# Autodesk Inventor assembly: Tower Pro MG90S Micro servo
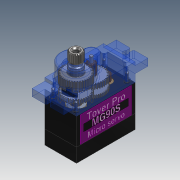
[picture p0: Inventor's stored thumbnail of the model, 180x180]
Saved by Autodesk Inventor 2017 (Build 210142000, 142)
## iProperties
Created: 2018-08-23
Part Number: Tower Pro MG90S Micro servo
Document SubType Name: Assembly
Designer: Shepelev
Mass: 15.118 g
Surface Area: 91.105 cm^2
Volume: 4.7278 cm^3
Density: 3.19769 g/cm^3
Author: Shepelev
## Documents named in this file (14)
- C:\Users\Anton\Desktop\Tower Pro MG90S Micro servo\Tower Pro MG90S Micro servo.iam
- C:\Users\Anton\Desktop\Tower Pro MG90S Micro servo\основание крпуса редуктора.ipt
- C:\Users\Anton\Desktop\Tower Pro MG90S Micro servo\Вал промежуточный.ipt
- C:\Users\Anton\Desktop\Tower Pro MG90S Micro servo\Вал последний с чем то.ipt
- C:\Users\Anton\Desktop\Tower Pro MG90S Micro servo\Моторчик.ipt
- C:\Users\Anton\Desktop\Tower Pro MG90S Micro servo\Tower Pro MG90S Micro servo\Мастер проектирования\Цилиндрическое зубчатое зацепление2.iam
- C:\Users\Anton\Desktop\Tower Pro MG90S Micro servo\Tower Pro MG90S Micro servo\Мастер проектирования\Цилиндрическое зубчатое зацепление3.iam
- C:\Users\Anton\Desktop\Tower Pro MG90S Micro servo\Tower Pro MG90S Micro servo\Мастер проектирования\Цилиндрическое зубчатое зацепление4.iam
- C:\Users\Anton\Desktop\Tower Pro MG90S Micro servo\Tower Pro MG90S Micro servo\Мастер проектирования\Цилиндрическое зубчатое зацепление5.iam
- C:\Users\Anton\Desktop\Tower Pro MG90S Micro servo\ограничитель.ipt
- C:\Users\Anton\Desktop\Tower Pro MG90S Micro servo\Крышка корпуса.ipt
- C:\Users\Anton\Desktop\Tower Pro MG90S Micro servo\Крышка корпуса задняя.ipt
- C:\Users\Anton\Desktop\Tower Pro MG90S Micro servo\Длинный винт.ipt
- C:\Users\Anton\Desktop\Tower Pro MG90S Micro servo\Этикетка.ipt
## Components (17 placed, 10 different names)
1. основание крпуса редуктора:1 — Совмещение:1, Заподлицо:1, Заподлицо:2, Вставка:1, Вставка:2, Вставка:3, Совмещение:2, Совмещение:4, Совмещение:6, Совмещение:23, Совмещение:24, Совмещение:25, Совмещение:26, Совмещение:27, Совмещение:28, Совмещение:29, Заподлицо:5, Заподлицо:6, Заподлицо:7, Заподлицо:8, Совмещение:30
2. Вал промежуточный:1 — Вставка:1, Заподлицо:3, Совмещение:5, Совмещение:7, Совмещение:14, Совмещение:18
3. Вал последний с чем то:1 — Вставка:2, Заподлицо:4, Совмещение:9, Совмещение:12, С поворотом:1
4. Моторчик:1 — Вставка:3, Совмещение:2, Совмещение:3
5. Цилиндрическое зубчатое зацепление:2 [sub-assembly] — Совмещение:3, Совмещение:4, Совмещение:5, Совмещение:6, Совмещение:8, Совмещение:10, Совмещение:11
6. Цилиндрическое зубчатое зацепление:3 [sub-assembly] — Совмещение:7, Совмещение:8, Совмещение:9, Совмещение:10, Совмещение:11, Совмещение:13, Совмещение:15, Совмещение:16
7. Цилиндрическое зубчатое зацепление:4 [sub-assembly] — Совмещение:12, Совмещение:13, Совмещение:14, Совмещение:15, Совмещение:16, Вставка:8, Совмещение:17, Совмещение:19
8. Цилиндрическое зубчатое зацепление:5 [sub-assembly] — Совмещение:18, Совмещение:19, Совмещение:20, Совмещение:21, Совмещение:22
9. ограничитель:2 — Вставка:8, Совмещение:17, С поворотом:1, Совмещение:20, Совмещение:21, Совмещение:22
10. Крышка корпуса:1 — Совмещение:23, Совмещение:24, Совмещение:25
11. Крышка корпуса задняя:1 — Совмещение:26, Совмещение:27, Совмещение:28, Вставка:9, Вставка:10, Вставка:11, Вставка:12
12. Длинный винт:1 — Вставка:9
13. Длинный винт:2 — Вставка:11
14. Длинный винт:3 — Вставка:10
15. Длинный винт:4 — Вставка:12
16. Этикетка:1 — Совмещение:29, Заподлицо:5, Заподлицо:6
17. Этикетка:2 — Заподлицо:7, Заподлицо:8, Совмещение:30
## Relationships (47: Mate 30, Flush 8, Insert 8, RevoluteJoint 1)
- Совмещение:1 [Mate]: основание крпуса редуктора:1
- Заподлицо:1 [Flush]: основание крпуса редуктора:1
- Заподлицо:2 [Flush]: основание крпуса редуктора:1
- Вставка:1 [Insert]: основание крпуса редуктора:1 ↔ Вал промежуточный:1
- Заподлицо:3 [Flush]: Вал промежуточный:1
- Вставка:2 [Insert]: основание крпуса редуктора:1 ↔ Вал последний с чем то:1
- Заподлицо:4 [Flush]: Вал последний с чем то:1
- Вставка:3 [Insert]: основание крпуса редуктора:1 ↔ Моторчик:1
- Совмещение:2 [Mate]: основание крпуса редуктора:1 ↔ Моторчик:1
- Совмещение:3 [Mate]: Моторчик:1 ↔ Цилиндрическое зубчатое зацепление:2
- Совмещение:4 [Mate]: основание крпуса редуктора:1 ↔ Цилиндрическое зубчатое зацепление:2
- Совмещение:5 [Mate]: Вал промежуточный:1 ↔ Цилиндрическое зубчатое зацепление:2
- Совмещение:6 [Mate]: основание крпуса редуктора:1 ↔ Цилиндрическое зубчатое зацепление:2
- Совмещение:7 [Mate]: Вал промежуточный:1 ↔ Цилиндрическое зубчатое зацепление:3
- Совмещение:8 [Mate]: Цилиндрическое зубчатое зацепление:2 ↔ Цилиндрическое зубчатое зацепление:3
- Совмещение:9 [Mate]: Вал последний с чем то:1 ↔ Цилиндрическое зубчатое зацепление:3
- Совмещение:10 [Mate]: Цилиндрическое зубчатое зацепление:2 ↔ Цилиндрическое зубчатое зацепление:3
- Совмещение:11 [Mate]: Цилиндрическое зубчатое зацепление:2 ↔ Цилиндрическое зубчатое зацепление:3
- Совмещение:12 [Mate]: Вал последний с чем то:1 ↔ Цилиндрическое зубчатое зацепление:4
- Совмещение:13 [Mate]: Цилиндрическое зубчатое зацепление:3 ↔ Цилиндрическое зубчатое зацепление:4
- Совмещение:14 [Mate]: Вал промежуточный:1 ↔ Цилиндрическое зубчатое зацепление:4
- Совмещение:15 [Mate]: Цилиндрическое зубчатое зацепление:3 ↔ Цилиндрическое зубчатое зацепление:4
- Совмещение:16 [Mate]: Цилиндрическое зубчатое зацепление:3 ↔ Цилиндрическое зубчатое зацепление:4
- Вставка:8 [Insert]: Цилиндрическое зубчатое зацепление:4 ↔ ограничитель:2
- Совмещение:17 [Mate]: Цилиндрическое зубчатое зацепление:4 ↔ ограничитель:2
- С поворотом:1 [RevoluteJoint] (0.4 mm): Вал последний с чем то:1 ↔ ограничитель:2
- Совмещение:18 [Mate]: Вал промежуточный:1 ↔ Цилиндрическое зубчатое зацепление:5
- Совмещение:19 [Mate]: Цилиндрическое зубчатое зацепление:4 ↔ Цилиндрическое зубчатое зацепление:5
- Совмещение:20 [Mate]: Цилиндрическое зубчатое зацепление:5 ↔ ограничитель:2
- Совмещение:21 [Mate]: Цилиндрическое зубчатое зацепление:5 ↔ ограничитель:2
- Совмещение:22 [Mate]: Цилиндрическое зубчатое зацепление:5 ↔ ограничитель:2
- Совмещение:23 [Mate]: основание крпуса редуктора:1 ↔ Крышка корпуса:1
- Совмещение:24 [Mate]: основание крпуса редуктора:1 ↔ Крышка корпуса:1
- Совмещение:25 [Mate]: основание крпуса редуктора:1 ↔ Крышка корпуса:1
- Совмещение:26 [Mate]: основание крпуса редуктора:1 ↔ Крышка корпуса задняя:1
- Совмещение:27 [Mate]: основание крпуса редуктора:1 ↔ Крышка корпуса задняя:1
- Совмещение:28 [Mate]: основание крпуса редуктора:1 ↔ Крышка корпуса задняя:1
- Вставка:9 [Insert]: Крышка корпуса задняя:1 ↔ Длинный винт:1
- Вставка:10 [Insert]: Крышка корпуса задняя:1 ↔ Длинный винт:3
- Вставка:11 [Insert]: Крышка корпуса задняя:1 ↔ Длинный винт:2
- Вставка:12 [Insert]: Крышка корпуса задняя:1 ↔ Длинный винт:4
- Совмещение:29 [Mate]: основание крпуса редуктора:1 ↔ Этикетка:1
- Заподлицо:5 [Flush] (1.5 mm): основание крпуса редуктора:1 ↔ Этикетка:1
- Заподлицо:6 [Flush] (0.25 mm): основание крпуса редуктора:1 ↔ Этикетка:1
- Заподлицо:7 [Flush] (0.25 mm): основание крпуса редуктора:1 ↔ Этикетка:2
- Заподлицо:8 [Flush] (1.5 mm): основание крпуса редуктора:1 ↔ Этикетка:2
- Совмещение:30 [Mate]: основание крпуса редуктора:1 ↔ Этикетка:2
